# Autodesk Inventor assembly: Spike_Assem
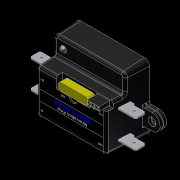
[picture p0: Inventor's stored thumbnail of the model, 180x180]
Saved by Autodesk Inventor 2012 (Build 160160000, 160)
## iProperties
Company: Team 801
Created: 2006-06-01
Part Number: Spike_Assem
Document SubType Name: Assembly
Designer: Jeffrey M
Catalog Web Link: www.team801.org
Mass: 42.1192 g
Surface Area: 102.966 cm^2
Volume: 42.1192 cm^3
Density: 1 g/cm^3
Author: Jeffrey M
## Documents named in this file (3)
- Z:\UserData\Documents\Inventor\team1885frc\Electronics\spike relay\Spike_Assem.iam
- Z:\UserData\Documents\Inventor\team1885frc\Electronics\spike relay\spike_relay.ipt
- Z:\UserData\Documents\Inventor\team1885frc\Electronics\spike relay\PMW_Terminal.ipt
## Components (2 placed, 2 different names)
1. spike_relay:1 — Mate:1, Mate:2, Mate:3
2. PMW_Terminal:1 — Mate:1, Mate:2, Mate:3
## Relationships (3: Mate 3)
- Mate:1: spike_relay:1 ↔ PMW_Terminal:1
- Mate:2: spike_relay:1 ↔ PMW_Terminal:1
- Mate:3: spike_relay:1 ↔ PMW_Terminal:1
